# Autodesk Inventor assembly: Mark 4.5
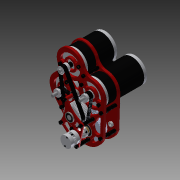
[picture p0: Inventor's stored thumbnail of the model, 180x180]
Saved by Autodesk Inventor 2013 (Build 170138000, 138)
## iProperties
Created: 2013-06-28
Part Number: Mark 4.5
Document SubType Name: Assembly
Designer: mvarma
Author: mvarma
## Documents named in this file (58)
- C:\Users\mvarma\Desktop\GRT 2013-2014 Gearbox\Mark 4\Mark 4.5.iam
- C:\Users\mvarma\Desktop\GRT 2013-2014 Gearbox\Mark 4\Plates\Mounting Plate.ipt
- C:\Users\mvarma\Desktop\GRT 2013-2014 Gearbox\Mark 4\Plates\Cim Plate.ipt
- C:\Users\mvarma\Desktop\GRT 2013-2014 Gearbox\Mark 4\Plates\Pnuematic Plate.ipt
- C:\Users\mvarma\Desktop\GRT 2013-2014 Gearbox\Mark 4\Plates\Main Connecting Standoff.ipt
- C:\Users\mvarma\Desktop\GRT 2013-2014 Gearbox\Mark 4\Pem Nuts\10-32 Clinch Style Pem Nut .091 Minimum Panel Thickness.ipt
- C:\Users\mvarma\Desktop\GRT 2013-2014 Gearbox\Mark 4\Pem Nuts\.25-20 Clinch Style Pem Nut .125 Minimum Panel Thickness.ipt
- C:\Users\mvarma\Desktop\GRT 2013-2014 Gearbox\Mark 4\Bearings\FR6-2ZZ - Hex.ipt
- C:\Users\mvarma\Desktop\GRT 2013-2014 Gearbox\Mark 4\Bearings\FR8-2RS.ipt
- C:\Users\mvarma\Desktop\GRT 2013-2014 Gearbox\Mark 4\Bearings\FR6-2RS.ipt
- C:\Users\mvarma\Desktop\GRT 2013-2014 Gearbox\Mark 4\Encoder\Encoder Mount.ipt
- C:\Users\mvarma\Desktop\GRT 2013-2014 Gearbox\Mark 4\Encoder\S4-120-250-N-S-B.ipt
- C:\Users\mvarma\Desktop\GRT 2013-2014 Gearbox\Mark 4\Shafts\Cluster Shaft.ipt
- C:\Users\mvarma\Desktop\GRT 2013-2014 Gearbox\Mark 4\Shafts\Flexible Shaft Coupler 6208K411.ipt
- C:\Users\mvarma\Desktop\GRT 2013-2014 Gearbox\Mark 4\Spacers\Cluster Shaft Spacer.ipt
- C:\Users\mvarma\Desktop\GRT 2013-2014 Gearbox\Mark 4\Gears\15T 20DP - .375 Hex Bore.ipt
- C:\Users\mvarma\Desktop\GRT 2013-2014 Gearbox\Mark 4\Gears\28T 20DP - .375 Hex Bore.ipt
- C:\Users\mvarma\Desktop\GRT 2013-2014 Gearbox\Mark 4\Shafts\Output Shaft.ipt
- C:\Users\mvarma\Desktop\GRT 2013-2014 Gearbox\Mark 4\Spacers\Shim 10 thou .500 Bore.ipt
- C:\Users\mvarma\Desktop\GRT 2013-2014 Gearbox\Mark 4\Bearings\R10-Open.ipt
- C:\Users\mvarma\Desktop\GRT 2013-2014 Gearbox\Mark 4\Gears\35T 20DP - .188 Ball Shifting Bore.ipt
- C:\Users\mvarma\Desktop\GRT 2013-2014 Gearbox\Mark 4\Gears\48T 20DP - .188 Ball Shifting Bore.ipt
- C:\Users\mvarma\Desktop\GRT 2013-2014 Gearbox\Mark 4\Bearings\Thrust Bearing Washer - .6250 Bore.ipt
- C:\Users\mvarma\Desktop\GRT 2013-2014 Gearbox\Mark 4\Spacers\Shim 10 thou .625 Bore.ipt
- C:\Users\mvarma\Desktop\GRT 2013-2014 Gearbox\Mark 4\Bolts\Socket Head Cap Screw 10-32 Thread 1.750 Length.ipt
- C:\Users\mvarma\Desktop\GRT 2013-2014 Gearbox\Mark 4\Plates\Supporting Plate Standoff.ipt
- C:\Users\mvarma\Desktop\GRT 2013-2014 Gearbox\Mark 4\Spacers\Shim 10 thou .375 Bore.ipt
- C:\Users\mvarma\Desktop\GRT 2013-2014 Gearbox\Mark 4\Pulleys\48T 3mm GT2 - .375 Hex Broach - Hubless.ipt
- C:\Users\mvarma\Desktop\GRT 2013-2014 Gearbox\Mark 4\Pem Nuts\4-40 Clinch Style Pem Nut .091 Minimum Panel Thickness.ipt
- C:\Users\mvarma\Desktop\GRT 2013-2014 Gearbox\Mark 4\Shafts\Tensioning Shaft.ipt
- C:\Users\mvarma\Desktop\GRT 2013-2014 Gearbox\Mark 4\Spacers\Belt Shaft Spacer 2.ipt
- C:\Users\mvarma\Desktop\GRT 2013-2014 Gearbox\Mark 4\Bearings\R4-2RS.ipt
- C:\Users\mvarma\Desktop\GRT 2013-2014 Gearbox\Mark 4\Bolts\Socket Head Cap Screw 10-32 Thread 1.500 Length.ipt
- C:\Users\mvarma\Desktop\GRT 2013-2014 Gearbox\Mark 4\Motors\CIM Can.ipt
- C:\Users\mvarma\Desktop\GRT 2013-2014 Gearbox\Mark 4\Motors\Mini CIM Can.ipt
- C:\Users\mvarma\Desktop\GRT 2013-2014 Gearbox\Mark 4\Motors\Rotor.ipt
- C:\Users\mvarma\Desktop\GRT 2013-2014 Gearbox\Mark 4\Bolts\Socket Head Cap Screw 10-32 Thread 3.000 Length.ipt
- C:\Users\mvarma\Desktop\GRT 2013-2014 Gearbox\Mark 4\Belts\267 mm Belt.ipt
- C:\Users\mvarma\Desktop\GRT 2013-2014 Gearbox\Mark 4\Belts\285 mm Belt.ipt
- C:\Users\mvarma\Desktop\GRT 2013-2014 Gearbox\Mark 4\Pulleys\16T 3mm GT2 - 8mm Key Broach.ipt
- C:\Users\mvarma\Desktop\GRT 2013-2014 Gearbox\Mark 4\Spacers\Cim Spacer.ipt
- C:\Users\mvarma\Desktop\GRT 2013-2014 Gearbox\Mark 4\Spacers\MiniCim Spacer.ipt
- C:\Users\mvarma\Desktop\GRT 2013-2014 Gearbox\Mark 4\Shafts\Ball Shifting Shaft.ipt
- C:\Users\mvarma\Desktop\GRT 2013-2014 Gearbox\Mark 4\Shafts\Output Shaft Insert.ipt
- C:\Users\mvarma\Desktop\GRT 2013-2014 Gearbox\Mark 4\Bearings\R3-2RS.ipt
- C:\Users\mvarma\Desktop\GRT 2013-2014 Gearbox\Mark 4\.0625 Spring Pin .2500 Long.ipt
- C:\Users\mvarma\Desktop\GRT 2013-2014 Gearbox\Mark 4\Pneumatic\Pneumatic Connector -Actuator Side.ipt
- C:\Users\mvarma\Desktop\GRT 2013-2014 Gearbox\Mark 4\Pneumatic\Pneumatic Connector -Shaft Side Cover.ipt
- C:\Users\mvarma\Desktop\GRT 2013-2014 Gearbox\Mark 4\Pneumatic\Pancake Pneumatic.iam
- C:\Users\mvarma\Desktop\GRT 2013-2014 Gearbox\Mark 4\Bolts\Button Head Cap Screw 4-40 Thread .125 Length.ipt
- C:\Users\mvarma\Desktop\GRT 2013-2014 Gearbox\Mark 4\Shafts\Output Shaft Hex Sleave.ipt
- C:\Users\mvarma\Desktop\GRT 2013-2014 Gearbox\Mark 4\Frame Segment.ipt
- C:\Users\mvarma\Desktop\GRT 2013-2014 Gearbox\Mark 4\Bolts\Socket Head Cap Screw 6-32 Thread 1.000 Length.ipt
- C:\Users\mvarma\Desktop\GRT 2013-2014 Gearbox\Mark 4\Plates\Cim Adjustment Block.ipt
- C:\Users\mvarma\Desktop\GRT 2013-2014 Gearbox\Mark 4\Bolts\Socket Head Cap Screw 6-32 Thread .500 Length.ipt
- C:\Users\mvarma\Desktop\GRT 2013-2014 Gearbox\Mark 4\Bolts\Socket Head Cap Screw 6-32 Thread .375 Length.ipt
- C:\Users\mvarma\Desktop\GRT 2013-2014 Gearbox\Mark 4\Bolts\Socket Head Cap Screw 10-32 Thread .750 Length.ipt
- C:\Users\mvarma\Desktop\GRT 2013-2014 Gearbox\Mark 4\Bolts\Socket Head Cap Screw 4-40 Thread 1.000 Length.ipt
## Components (110 placed, 57 different names)
1. Frame Segment:1 — Mate:228, Mate:229
2. Socket Head Cap Screw 4-40 Thread 1.000 Length:1 — Mate:270, Mate:272
3. Socket Head Cap Screw 4-40 Thread 1.000 Length:2 — Mate:271, Mate:273
4. 267 mm Belt:1 — Mate:174, Mate:175, Mate:179, Flush:2, Flush:3
5. 285 mm Belt:1 — Mate:176, Mate:177, Mate:178, Flush:1
6. Socket Head Cap Screw 6-32 Thread 1.000 Length:1 — Mate:232, Mate:234
7. Socket Head Cap Screw 6-32 Thread 1.000 Length:2 — Mate:231, Mate:233
8. S4-120-250-N-S-B:1 — Mate:66, Mate:67
9. Flexible Shaft Coupler 6208K411:1 — Mate:64, Mate:65, Mate:66, Mate:67
10. Encoder Mount:1 — Mate:225, Mate:226, Mate:227, Mate:231, Mate:232, Mate:233, Mate:234
11. Cim Spacer:1 — Mate:184, Mate:185
12. MiniCim Spacer:1 — Mate:187, Mate:188
13. Cim Spacer:2 — Mate:183, Mate:186
14. CIM Can:1 — Mate:153, Mate:154, Mate:155, Mate:163, Mate:166, Mate:185
15. CIM Can:2 — Mate:156, Mate:157, Mate:158, Mate:164, Mate:165, Mate:186
16. Mini CIM Can:1 — Mate:159, Mate:160, Mate:161, Mate:162, Mate:167, Mate:188, Mate:254
17. Rotor:1 — Mate:164, Mate:165, Mate:175, Mate:181, Mate:183
18. Rotor:2 — Mate:163, Mate:166, Mate:180, Mate:184
19. Rotor:3 — Mate:162, Mate:167, Mate:177, Mate:182, Mate:187
20. Socket Head Cap Screw 10-32 Thread .750 Length:1 — Mate:262, Mate:263
21. Socket Head Cap Screw 10-32 Thread .750 Length:2 — Mate:252, Mate:253
22. Socket Head Cap Screw 10-32 Thread .750 Length:3 — Mate:254, Mate:255
23. Socket Head Cap Screw 10-32 Thread .750 Length:4 — Mate:260, Mate:261
24. Socket Head Cap Screw 10-32 Thread .750 Length:5 — Mate:256, Mate:259
25. Socket Head Cap Screw 10-32 Thread .750 Length:6 — Mate:257, Mate:258
26. Pneumatic Connector -Actuator Side:1 — Mate:196, Mate:197, Mate:198, Mate:203, Mate:210, Mate:211
27. Pneumatic Connector -Shaft Side Cover:1 — Mate:196, Mate:197, Mate:198, Mate:201, Mate:214, Mate:219, Mate:220, Mate:221, Mate:222
28. Pancake Pneumatic:1 [sub-assembly] — Mate:209, Mate:210, Mate:211, Mate:212, Mate:213, Mate:270, Mate:271, Mate:272, Mate:273
29. Button Head Cap Screw 4-40 Thread .125 Length:1 — Mate:221, Mate:222
30. Button Head Cap Screw 4-40 Thread .125 Length:2 — Mate:219, Mate:220
31. 16T 3mm GT2 - 8mm Key Broach:1 — Mate:180, Flush:3
32. 16T 3mm GT2 - 8mm Key Broach:2 — Mate:181, Flush:2
33. 16T 3mm GT2 - 8mm Key Broach:3 — Mate:182, Flush:1
34. Supporting Plate Standoff:1 — Mate:117, Mate:120, Mate:122
35. Supporting Plate Standoff:2 — Mate:118, Mate:121
36. Supporting Plate Standoff:3 — Mate:116, Mate:119
37. Main Connecting Standoff:1 — Mate:10, Mate:28
38. Main Connecting Standoff:2 — Mate:11, Mate:29
39. Main Connecting Standoff:3 — Mate:3, Mate:12, Mate:27, Mate:140
40. Main Connecting Standoff:4 — Mate:15, Mate:26
41. Main Connecting Standoff:5 — Mate:5, Mate:16, Mate:25
42. Main Connecting Standoff:6 — Mate:17, Mate:23
43. Main Connecting Standoff:7 — Mate:20, Mate:21
44. Main Connecting Standoff:8 — Mate:8, Mate:19, Mate:24
45. Main Connecting Standoff:9 — Mate:18, Mate:22, Mate:206
46. Mounting Plate:1 — Mate:3, Mate:5, Mate:8, Mate:21, Mate:22, Mate:23, Mate:24, Mate:25, Mate:26, Mate:27, Mate:28, Mate:29, Mate:31, Mate:34, Mate:36, Mate:39, Mate:40, Mate:41, Mate:42, Mate:43, Mate:44, Mate:45, Mate:46, Mate:47, Mate:48, Mate:49, Mate:50, Mate:51, Mate:53, Mate:55, Mate:56, Mate:57, Mate:68, Mate:73, Mate:74, Mate:225, Mate:226, Mate:227, Mate:229, Mate:235, Mate:236, Mate:237, Mate:243, Mate:244, Mate:245, Mate:264, Mate:265, Mate:266, Mate:267, Mate:268, Mate:269
47. FR8-2RS:1 — Mate:53, Mate:55, Mate:80, Mate:83
48. FR6-2RS:1 — Mate:56, Mate:57, Mate:72
49. Cim Plate:1 — Mate:10, Mate:11, Mate:12, Mate:15, Mate:16, Mate:17, Mate:18, Mate:19, Mate:20, Mate:58, Mate:59, Mate:60, Mate:61, Mate:102, Mate:103, Mate:104, Mate:105, Mate:106, Mate:107, Mate:108, Mate:109, Mate:110, Mate:111, Mate:112, Mate:113, Mate:114, Mate:115, Mate:116, Mate:117, Mate:118, Mate:119, Mate:120, Mate:121, Mate:139, Mate:140, Mate:141, Mate:142, Mate:153, Mate:154, Mate:155, Mate:156, Mate:157, Mate:158, Mate:159, Mate:160, Mate:161, Mate:174, Mate:176, Mate:206, Mate:252, Mate:253, Mate:255, Mate:256, Mate:257, Mate:258, Mate:259, Mate:260, Mate:261, Mate:262, Mate:263
50. FR6-2ZZ - Hex:1 — Mate:60, Mate:61, Mate:79, Mate:125
51. FR8-2RS:2 — Mate:58, Mate:59, Mate:214
52. Socket Head Cap Screw 10-32 Thread 1.500 Length:1 — Mate:151, Mate:152
53. Pnuematic Plate:1 — Mate:114, Mate:115, Mate:122, Mate:133, Mate:134, Mate:139, Mate:146, Mate:151, Mate:152, Mate:168, Mate:169, Mate:170, Mate:171, Mate:172, Mate:173, Mate:209, Mate:212, Mate:213, Mate:215, Mate:216, Mate:217, Mate:218
54. FR6-2RS:2 — Mate:133, Mate:134
55. Socket Head Cap Screw 10-32 Thread 3.000 Length:1 — Mate:170, Mate:173
56. Socket Head Cap Screw 10-32 Thread 3.000 Length:2 — Mate:169, Mate:171
57. Socket Head Cap Screw 10-32 Thread 3.000 Length:3 — Mate:168, Mate:172
58. Ball Shifting Shaft:1 — Mate:191, Mate:192, Mate:193, Mate:194, Mate:195, Mate:201
59. R3-2RS:1 — Mate:192, Mate:193, Mate:203
60. .0625 Spring Pin .2500 Long:1 — Mate:194, Mate:195
61. Cluster Shaft:1 — Mate:64, Mate:65, Mate:68, Mate:71, Mate:75, Mate:76, Mate:79, Mate:123, Mate:124, Mate:126, Mate:127, Mate:128, Mate:129
62. Cluster Shaft Spacer:1 — Mate:71, Mate:72, Mate:78
63. 15T 20DP - .375 Hex Bore:1 — Mate:74, Mate:76, Mate:77
64. 28T 20DP - .375 Hex Bore:1 — Mate:73, Mate:75, Mate:77, Mate:78
65. Shim 10 thou .375 Bore:1 — Mate:123, Mate:132
66. Shim 10 thou .500 Bore:2 — Mate:124, Mate:125, Mate:131
67. 48T 3mm GT2 - .375 Hex Broach - Hubless:1 — Mate:126, Mate:128, Mate:130, Mate:132, Mate:178
68. 48T 3mm GT2 - .375 Hex Broach - Hubless:2 — Mate:127, Mate:129, Mate:130, Mate:131, Mate:179
69. Output Shaft Insert:1 — Mate:189, Mate:190, Mate:191
70. Shim 10 thou .625 Bore:1 — Mate:96, Mate:97
71. Thrust Bearing Washer - .6250 Bore:2 — Mate:94, Mate:95, Mate:97
72. 48T 20DP - .188 Ball Shifting Bore:1 — Mate:92, Mate:93, Mate:95
73. R10-Open:1 — Mate:90, Mate:91, Mate:93
74. Thrust Bearing Washer - .6250 Bore:1 — Mate:88, Mate:89, Mate:91
75. 35T 20DP - .188 Ball Shifting Bore:1 — Mate:86, Mate:87, Mate:89
76. R10-Open:2 — Mate:84, Mate:85, Mate:87
77. Shim 10 thou .500 Bore:1 — Mate:81, Mate:82, Mate:83, Mate:85
78. Output Shaft:1 — Mate:80, Mate:81, Mate:82, Mate:84, Mate:86, Mate:88, Mate:90, Mate:92, Mate:94, Mate:96, Mate:189, Mate:190, Mate:223, Mate:224, Flush:4, Mate:228
79. Output Shaft Hex Sleave:1 — Mate:223, Mate:224, Flush:4
80. Tensioning Shaft:1 — Mate:141, Mate:142, Mate:143, Mate:149
81. Belt Shaft Spacer 2:1 — Mate:143, Mate:146, Mate:150
82. R4-2RS:1 — Mate:147, Mate:148, Mate:149, Mate:150
83. R4-2RS:2 — Mate:147, Mate:148
84. Cim Adjustment Block:1 — Mate:235, Mate:236, Mate:237, Mate:238, Mate:239, Mate:240, Mate:241, Mate:251
85. Cim Adjustment Block:2 — Mate:243, Mate:244, Mate:245, Mate:246, Mate:247, Mate:248, Mate:249, Mate:250
86. Socket Head Cap Screw 6-32 Thread .500 Length:1 — Mate:239, Mate:240
87. Socket Head Cap Screw 6-32 Thread .500 Length:2 — Mate:238, Mate:241
88. Socket Head Cap Screw 6-32 Thread .375 Length:2 — Mate:251
89. Socket Head Cap Screw 6-32 Thread .500 Length:4 — Mate:246, Mate:249
90. Socket Head Cap Screw 6-32 Thread .500 Length:5 — Mate:247, Mate:248
91. Socket Head Cap Screw 6-32 Thread .375 Length:1 — Mate:250
92. 10-32 Clinch Style Pem Nut .091 Minimum Panel Thickness:1 — Mate:41, Mate:268
93. 10-32 Clinch Style Pem Nut .091 Minimum Panel Thickness:2 — Mate:34, Mate:40
94. 10-32 Clinch Style Pem Nut .091 Minimum Panel Thickness:3 — Mate:39, Mate:267
95. 10-32 Clinch Style Pem Nut .091 Minimum Panel Thickness:4 — Mate:31, Mate:42
96. 10-32 Clinch Style Pem Nut .091 Minimum Panel Thickness:5 — Mate:43, Mate:266
97. 10-32 Clinch Style Pem Nut .091 Minimum Panel Thickness:6 — Mate:44, Mate:265
98. 10-32 Clinch Style Pem Nut .091 Minimum Panel Thickness:7 — Mate:47, Mate:269
99. 10-32 Clinch Style Pem Nut .091 Minimum Panel Thickness:8 — Mate:36, Mate:45
100. 10-32 Clinch Style Pem Nut .091 Minimum Panel Thickness:9 — Mate:46, Mate:264
101. .25-20 Clinch Style Pem Nut .125 Minimum Panel Thickness:1 — Mate:49, Mate:50
102. .25-20 Clinch Style Pem Nut .125 Minimum Panel Thickness:2 — Mate:48, Mate:51
103. Socket Head Cap Screw 10-32 Thread 1.750 Length:4 — Mate:108, Mate:109
104. Socket Head Cap Screw 10-32 Thread 1.750 Length:5 — Mate:111, Mate:113
105. Socket Head Cap Screw 10-32 Thread 1.750 Length:6 — Mate:110, Mate:112
106. Socket Head Cap Screw 10-32 Thread 1.750 Length:7 — Mate:105, Mate:106
107. Socket Head Cap Screw 10-32 Thread 1.750 Length:8 — Mate:104, Mate:107
108. Socket Head Cap Screw 10-32 Thread 1.750 Length:9 — Mate:102, Mate:103
109. 4-40 Clinch Style Pem Nut .091 Minimum Panel Thickness:1 — Mate:216, Mate:218
110. 4-40 Clinch Style Pem Nut .091 Minimum Panel Thickness:2 — Mate:215, Mate:217
## Relationships (240: Mate 234, Flush 4, Tangent 2)
- Mate:3: Main Connecting Standoff:3 ↔ Mounting Plate:1
- Mate:5: Main Connecting Standoff:5 ↔ Mounting Plate:1
- Mate:8: Main Connecting Standoff:8 ↔ Mounting Plate:1
- Mate:10: Main Connecting Standoff:1 ↔ Cim Plate:1
- Mate:11: Main Connecting Standoff:2 ↔ Cim Plate:1
- Mate:12: Main Connecting Standoff:3 ↔ Cim Plate:1
- Mate:15: Main Connecting Standoff:4 ↔ Cim Plate:1
- Mate:16: Main Connecting Standoff:5 ↔ Cim Plate:1
- Mate:17: Main Connecting Standoff:6 ↔ Cim Plate:1
- Mate:18: Main Connecting Standoff:9 ↔ Cim Plate:1
- Mate:19: Main Connecting Standoff:8 ↔ Cim Plate:1
- Mate:20: Main Connecting Standoff:7 ↔ Cim Plate:1
- Mate:21: Main Connecting Standoff:7 ↔ Mounting Plate:1
- Mate:22: Main Connecting Standoff:9 ↔ Mounting Plate:1
- Mate:23: Main Connecting Standoff:6 ↔ Mounting Plate:1
- Mate:24: Main Connecting Standoff:8 ↔ Mounting Plate:1
- Mate:25: Main Connecting Standoff:5 ↔ Mounting Plate:1
- Mate:26: Main Connecting Standoff:4 ↔ Mounting Plate:1
- Mate:27: Main Connecting Standoff:3 ↔ Mounting Plate:1
- Mate:28: Main Connecting Standoff:1 ↔ Mounting Plate:1
- Mate:29: Main Connecting Standoff:2 ↔ Mounting Plate:1
- Mate:31: Mounting Plate:1 ↔ 10-32 Clinch Style Pem Nut .091 Minimum Panel Thickness:4
- Mate:34: Mounting Plate:1 ↔ 10-32 Clinch Style Pem Nut .091 Minimum Panel Thickness:2
- Mate:36: Mounting Plate:1 ↔ 10-32 Clinch Style Pem Nut .091 Minimum Panel Thickness:8
- Mate:39: Mounting Plate:1 ↔ 10-32 Clinch Style Pem Nut .091 Minimum Panel Thickness:3
- Mate:40: Mounting Plate:1 ↔ 10-32 Clinch Style Pem Nut .091 Minimum Panel Thickness:2
- Mate:41: Mounting Plate:1 ↔ 10-32 Clinch Style Pem Nut .091 Minimum Panel Thickness:1
- Mate:42: Mounting Plate:1 ↔ 10-32 Clinch Style Pem Nut .091 Minimum Panel Thickness:4
- Mate:43: Mounting Plate:1 ↔ 10-32 Clinch Style Pem Nut .091 Minimum Panel Thickness:5
- Mate:44: Mounting Plate:1 ↔ 10-32 Clinch Style Pem Nut .091 Minimum Panel Thickness:6
- Mate:45: Mounting Plate:1 ↔ 10-32 Clinch Style Pem Nut .091 Minimum Panel Thickness:8
- Mate:46: Mounting Plate:1 ↔ 10-32 Clinch Style Pem Nut .091 Minimum Panel Thickness:9
- Mate:47: Mounting Plate:1 ↔ 10-32 Clinch Style Pem Nut .091 Minimum Panel Thickness:7
- Mate:48: Mounting Plate:1 ↔ .25-20 Clinch Style Pem Nut .125 Minimum Panel Thickness:2
- Mate:49: Mounting Plate:1 ↔ .25-20 Clinch Style Pem Nut .125 Minimum Panel Thickness:1
- Mate:50: Mounting Plate:1 ↔ .25-20 Clinch Style Pem Nut .125 Minimum Panel Thickness:1
- Mate:51: Mounting Plate:1 ↔ .25-20 Clinch Style Pem Nut .125 Minimum Panel Thickness:2
- Mate:53: Mounting Plate:1 ↔ FR8-2RS:1
- Mate:55: Mounting Plate:1 ↔ FR8-2RS:1
- Mate:56: Mounting Plate:1 ↔ FR6-2RS:1
- Mate:57: Mounting Plate:1 ↔ FR6-2RS:1
- Mate:58: Cim Plate:1 ↔ FR8-2RS:2
- Mate:59: Cim Plate:1 ↔ FR8-2RS:2
- Mate:60: Cim Plate:1 ↔ FR6-2ZZ - Hex:1
- Mate:61: Cim Plate:1 ↔ FR6-2ZZ - Hex:1
- Mate:64: Flexible Shaft Coupler 6208K411:1 ↔ Cluster Shaft:1
- Mate:65: Flexible Shaft Coupler 6208K411:1 ↔ Cluster Shaft:1
- Mate:66: S4-120-250-N-S-B:1 ↔ Flexible Shaft Coupler 6208K411:1
- Mate:67: S4-120-250-N-S-B:1 ↔ Flexible Shaft Coupler 6208K411:1
- Mate:68: Mounting Plate:1 ↔ Cluster Shaft:1
- Mate:71: Cluster Shaft:1 ↔ Cluster Shaft Spacer:1
- Mate:72: FR6-2RS:1 ↔ Cluster Shaft Spacer:1
- Mate:73: Mounting Plate:1 ↔ 28T 20DP - .375 Hex Bore:1
- Mate:74: Mounting Plate:1 ↔ 15T 20DP - .375 Hex Bore:1
- Mate:75: Cluster Shaft:1 ↔ 28T 20DP - .375 Hex Bore:1
- Mate:76: Cluster Shaft:1 ↔ 15T 20DP - .375 Hex Bore:1
- Mate:77: 15T 20DP - .375 Hex Bore:1 ↔ 28T 20DP - .375 Hex Bore:1
- Mate:78: Cluster Shaft Spacer:1 ↔ 28T 20DP - .375 Hex Bore:1
- Mate:79: FR6-2ZZ - Hex:1 ↔ Cluster Shaft:1
- Mate:80: FR8-2RS:1 ↔ Output Shaft:1
- Mate:81: Shim 10 thou .500 Bore:1 ↔ Output Shaft:1
- Mate:82: Shim 10 thou .500 Bore:1 ↔ Output Shaft:1
- Mate:83: FR8-2RS:1 ↔ Shim 10 thou .500 Bore:1
- Mate:84: R10-Open:2 ↔ Output Shaft:1
- Mate:85: R10-Open:2 ↔ Shim 10 thou .500 Bore:1
- Mate:86: 35T 20DP - .188 Ball Shifting Bore:1 ↔ Output Shaft:1
- Mate:87: 35T 20DP - .188 Ball Shifting Bore:1 ↔ R10-Open:2
- Mate:88: Thrust Bearing Washer - .6250 Bore:1 ↔ Output Shaft:1
- Mate:89: Thrust Bearing Washer - .6250 Bore:1 ↔ 35T 20DP - .188 Ball Shifting Bore:1
- Mate:90: R10-Open:1 ↔ Output Shaft:1
- Mate:91: R10-Open:1 ↔ Thrust Bearing Washer - .6250 Bore:1
- Mate:92: 48T 20DP - .188 Ball Shifting Bore:1 ↔ Output Shaft:1
- Mate:93: 48T 20DP - .188 Ball Shifting Bore:1 ↔ R10-Open:1
- Mate:94: Thrust Bearing Washer - .6250 Bore:2 ↔ Output Shaft:1
- Mate:95: Thrust Bearing Washer - .6250 Bore:2 ↔ 48T 20DP - .188 Ball Shifting Bore:1
- Mate:96: Shim 10 thou .625 Bore:1 ↔ Output Shaft:1
- Mate:97: Shim 10 thou .625 Bore:1 ↔ Thrust Bearing Washer - .6250 Bore:2
- Mate:102: Cim Plate:1 ↔ Socket Head Cap Screw 10-32 Thread 1.750 Length:9
- Mate:103: Cim Plate:1 ↔ Socket Head Cap Screw 10-32 Thread 1.750 Length:9
- Mate:104: Cim Plate:1 ↔ Socket Head Cap Screw 10-32 Thread 1.750 Length:8
- Mate:105: Cim Plate:1 ↔ Socket Head Cap Screw 10-32 Thread 1.750 Length:7
- Mate:106: Cim Plate:1 ↔ Socket Head Cap Screw 10-32 Thread 1.750 Length:7
- Mate:107: Cim Plate:1 ↔ Socket Head Cap Screw 10-32 Thread 1.750 Length:8
- Mate:108: Cim Plate:1 ↔ Socket Head Cap Screw 10-32 Thread 1.750 Length:4
- Mate:109: Cim Plate:1 ↔ Socket Head Cap Screw 10-32 Thread 1.750 Length:4
- Mate:110: Cim Plate:1 ↔ Socket Head Cap Screw 10-32 Thread 1.750 Length:6
- Mate:111: Cim Plate:1 ↔ Socket Head Cap Screw 10-32 Thread 1.750 Length:5
- Mate:112: Cim Plate:1 ↔ Socket Head Cap Screw 10-32 Thread 1.750 Length:6
- Mate:113: Cim Plate:1 ↔ Socket Head Cap Screw 10-32 Thread 1.750 Length:5
- Mate:114: Cim Plate:1 ↔ Pnuematic Plate:1
- Mate:115: Cim Plate:1 ↔ Pnuematic Plate:1
- Mate:116: Supporting Plate Standoff:3 ↔ Cim Plate:1
- Mate:117: Supporting Plate Standoff:1 ↔ Cim Plate:1
- Mate:118: Supporting Plate Standoff:2 ↔ Cim Plate:1
- Mate:119: Supporting Plate Standoff:3 ↔ Cim Plate:1
- Mate:120: Supporting Plate Standoff:1 ↔ Cim Plate:1
- Mate:121: Supporting Plate Standoff:2 ↔ Cim Plate:1
- Mate:122: Supporting Plate Standoff:1 ↔ Pnuematic Plate:1
- Mate:123: Cluster Shaft:1 ↔ Shim 10 thou .375 Bore:1
- Mate:124: Cluster Shaft:1 ↔ Shim 10 thou .500 Bore:2
- Mate:125: FR6-2ZZ - Hex:1 ↔ Shim 10 thou .500 Bore:2
- Mate:126: Cluster Shaft:1 ↔ 48T 3mm GT2 - .375 Hex Broach - Hubless:1
- Mate:127: Cluster Shaft:1 ↔ 48T 3mm GT2 - .375 Hex Broach - Hubless:2
- Mate:128: Cluster Shaft:1 ↔ 48T 3mm GT2 - .375 Hex Broach - Hubless:1
- Mate:129: Cluster Shaft:1 ↔ 48T 3mm GT2 - .375 Hex Broach - Hubless:2
- Mate:130: 48T 3mm GT2 - .375 Hex Broach - Hubless:1 ↔ 48T 3mm GT2 - .375 Hex Broach - Hubless:2
- Mate:131: Shim 10 thou .500 Bore:2 ↔ 48T 3mm GT2 - .375 Hex Broach - Hubless:2
- Mate:132: Shim 10 thou .375 Bore:1 ↔ 48T 3mm GT2 - .375 Hex Broach - Hubless:1
- Mate:133: Pnuematic Plate:1 ↔ FR6-2RS:2
- Mate:134: Pnuematic Plate:1 ↔ FR6-2RS:2
- Mate:139: Cim Plate:1 ↔ Pnuematic Plate:1
- Mate:140: Main Connecting Standoff:3 ↔ Cim Plate:1
- Mate:141: Cim Plate:1 ↔ Tensioning Shaft:1
- Mate:142: Cim Plate:1 ↔ Tensioning Shaft:1
- Mate:143: Tensioning Shaft:1 ↔ Belt Shaft Spacer 2:1
- Mate:146: Pnuematic Plate:1 ↔ Belt Shaft Spacer 2:1
- Mate:147: R4-2RS:1 ↔ R4-2RS:2
- Mate:148: R4-2RS:1 ↔ R4-2RS:2
- Mate:149: Tensioning Shaft:1 ↔ R4-2RS:1
- Mate:150: Belt Shaft Spacer 2:1 ↔ R4-2RS:1
- Mate:151: Socket Head Cap Screw 10-32 Thread 1.500 Length:1 ↔ Pnuematic Plate:1
- Mate:152: Socket Head Cap Screw 10-32 Thread 1.500 Length:1 ↔ Pnuematic Plate:1
- Mate:153: CIM Can:1 ↔ Cim Plate:1
- Mate:154: CIM Can:1 ↔ Cim Plate:1
- Mate:155: CIM Can:1 ↔ Cim Plate:1
- Mate:156: CIM Can:2 ↔ Cim Plate:1
- Mate:157: CIM Can:2 ↔ Cim Plate:1
- Mate:158: CIM Can:2 ↔ Cim Plate:1
- Mate:159: Mini CIM Can:1 ↔ Cim Plate:1
- Mate:160: Mini CIM Can:1 ↔ Cim Plate:1
- Mate:161: Mini CIM Can:1 ↔ Cim Plate:1
- Mate:162: Mini CIM Can:1 ↔ Rotor:3
- Mate:163: CIM Can:1 ↔ Rotor:2
- Mate:164: CIM Can:2 ↔ Rotor:1
- Mate:165: CIM Can:2 ↔ Rotor:1
- Mate:166: CIM Can:1 ↔ Rotor:2
- Mate:167: Mini CIM Can:1 ↔ Rotor:3
- Mate:168: Pnuematic Plate:1 ↔ Socket Head Cap Screw 10-32 Thread 3.000 Length:3
- Mate:169: Pnuematic Plate:1 ↔ Socket Head Cap Screw 10-32 Thread 3.000 Length:2
- Mate:170: Pnuematic Plate:1 ↔ Socket Head Cap Screw 10-32 Thread 3.000 Length:1
- Mate:171: Pnuematic Plate:1 ↔ Socket Head Cap Screw 10-32 Thread 3.000 Length:2
- Mate:172: Pnuematic Plate:1 ↔ Socket Head Cap Screw 10-32 Thread 3.000 Length:3
- Mate:173: Pnuematic Plate:1 ↔ Socket Head Cap Screw 10-32 Thread 3.000 Length:1
- Mate:174: 267 mm Belt:1 ↔ Cim Plate:1
- Mate:175: 267 mm Belt:1 ↔ Rotor:1
- Mate:176: 285 mm Belt:1 ↔ Cim Plate:1
- Mate:177: 285 mm Belt:1 ↔ Rotor:3
- Mate:178: 285 mm Belt:1 ↔ 48T 3mm GT2 - .375 Hex Broach - Hubless:1
- Mate:179: 267 mm Belt:1 ↔ 48T 3mm GT2 - .375 Hex Broach - Hubless:2
- Mate:180: Rotor:2 ↔ 16T 3mm GT2 - 8mm Key Broach:1
- Mate:181: Rotor:1 ↔ 16T 3mm GT2 - 8mm Key Broach:2
- Mate:182: Rotor:3 ↔ 16T 3mm GT2 - 8mm Key Broach:3
- Flush:1: 285 mm Belt:1 ↔ 16T 3mm GT2 - 8mm Key Broach:3
- Flush:2: 267 mm Belt:1 ↔ 16T 3mm GT2 - 8mm Key Broach:2
- Flush:3: 267 mm Belt:1 ↔ 16T 3mm GT2 - 8mm Key Broach:1
- Mate:183: Cim Spacer:2 ↔ Rotor:1
- Mate:184: Cim Spacer:1 ↔ Rotor:2
- Mate:185: Cim Spacer:1 ↔ CIM Can:1
- Mate:186: Cim Spacer:2 ↔ CIM Can:2
- Mate:187: MiniCim Spacer:1 ↔ Rotor:3
- Mate:188: MiniCim Spacer:1 ↔ Mini CIM Can:1
- Mate:189: Output Shaft Insert:1 ↔ Output Shaft:1
- Mate:190: Output Shaft Insert:1 ↔ Output Shaft:1
- Mate:191: Ball Shifting Shaft:1 ↔ Output Shaft Insert:1
- Mate:192: Ball Shifting Shaft:1 ↔ R3-2RS:1
- Mate:193: Ball Shifting Shaft:1 ↔ R3-2RS:1
- Mate:194: Ball Shifting Shaft:1 ↔ .0625 Spring Pin .2500 Long:1
- Mate:195: Ball Shifting Shaft:1 ↔ .0625 Spring Pin .2500 Long:1
- Mate:196: Pneumatic Connector -Actuator Side:1 ↔ Pneumatic Connector -Shaft Side Cover:1
- Mate:197: Pneumatic Connector -Actuator Side:1 ↔ Pneumatic Connector -Shaft Side Cover:1
- Mate:198: Pneumatic Connector -Actuator Side:1 ↔ Pneumatic Connector -Shaft Side Cover:1
- Mate:201: Pneumatic Connector -Shaft Side Cover:1 ↔ Ball Shifting Shaft:1
- Mate:203: Pneumatic Connector -Actuator Side:1 ↔ R3-2RS:1
- Mate:206: Main Connecting Standoff:9 ↔ Cim Plate:1
- Mate:209: Pancake Pneumatic:1 ↔ Pnuematic Plate:1
- Mate:210: Pneumatic Connector -Actuator Side:1 ↔ Pancake Pneumatic:1
- Mate:211: Pneumatic Connector -Actuator Side:1 ↔ Pancake Pneumatic:1
- Mate:212: Pancake Pneumatic:1 ↔ Pnuematic Plate:1
- Mate:213: Pancake Pneumatic:1 ↔ Pnuematic Plate:1
- Mate:214 (8.8582 mm): Pneumatic Connector -Shaft Side Cover:1 ↔ FR8-2RS:2
- Mate:215: Pnuematic Plate:1 ↔ 4-40 Clinch Style Pem Nut .091 Minimum Panel Thickness:2
- Mate:216: Pnuematic Plate:1 ↔ 4-40 Clinch Style Pem Nut .091 Minimum Panel Thickness:1
- Mate:217: Pnuematic Plate:1 ↔ 4-40 Clinch Style Pem Nut .091 Minimum Panel Thickness:2
- Mate:218: Pnuematic Plate:1 ↔ 4-40 Clinch Style Pem Nut .091 Minimum Panel Thickness:1
- Mate:219: Pneumatic Connector -Shaft Side Cover:1 ↔ Button Head Cap Screw 4-40 Thread .125 Length:2
- Mate:220: Pneumatic Connector -Shaft Side Cover:1 ↔ Button Head Cap Screw 4-40 Thread .125 Length:2
- Mate:221: Pneumatic Connector -Shaft Side Cover:1 ↔ Button Head Cap Screw 4-40 Thread .125 Length:1
- Mate:222: Pneumatic Connector -Shaft Side Cover:1 ↔ Button Head Cap Screw 4-40 Thread .125 Length:1
- Mate:223: Output Shaft:1 ↔ Output Shaft Hex Sleave:1
- Mate:224: Output Shaft:1 ↔ Output Shaft Hex Sleave:1
- Flush:4: Output Shaft:1 ↔ Output Shaft Hex Sleave:1
- Mate:225: Encoder Mount:1 ↔ Mounting Plate:1
- Mate:226: Encoder Mount:1 ↔ Mounting Plate:1
- Mate:227: Encoder Mount:1 ↔ Mounting Plate:1
- Mate:228: Frame Segment:1 ↔ Output Shaft:1
- Mate:229: Frame Segment:1 ↔ Mounting Plate:1
- Mate:231: Socket Head Cap Screw 6-32 Thread 1.000 Length:2 ↔ Encoder Mount:1
- Mate:232: Socket Head Cap Screw 6-32 Thread 1.000 Length:1 ↔ Encoder Mount:1
- Mate:233: Socket Head Cap Screw 6-32 Thread 1.000 Length:2 ↔ Encoder Mount:1
- Mate:234: Socket Head Cap Screw 6-32 Thread 1.000 Length:1 ↔ Encoder Mount:1
- Mate:235: Mounting Plate:1 ↔ Cim Adjustment Block:1
- Mate:236: Mounting Plate:1 ↔ Cim Adjustment Block:1
- Mate:237: Mounting Plate:1 ↔ Cim Adjustment Block:1
- Mate:238: Cim Adjustment Block:1 ↔ Socket Head Cap Screw 6-32 Thread .500 Length:2
- Mate:239: Cim Adjustment Block:1 ↔ Socket Head Cap Screw 6-32 Thread .500 Length:1
- Mate:240: Cim Adjustment Block:1 ↔ Socket Head Cap Screw 6-32 Thread .500 Length:1
- Mate:241: Cim Adjustment Block:1 ↔ Socket Head Cap Screw 6-32 Thread .500 Length:2
- [Tangent]: CIM Can:2 ↔ Socket Head Cap Screw 6-32 Thread .375 Length:2
- Mate:243: Mounting Plate:1 ↔ Cim Adjustment Block:2
- Mate:244: Mounting Plate:1 ↔ Cim Adjustment Block:2
- Mate:245: Mounting Plate:1 ↔ Cim Adjustment Block:2
- Mate:246: Cim Adjustment Block:2 ↔ Socket Head Cap Screw 6-32 Thread .500 Length:4
- Mate:247: Cim Adjustment Block:2 ↔ Socket Head Cap Screw 6-32 Thread .500 Length:5
- Mate:248: Cim Adjustment Block:2 ↔ Socket Head Cap Screw 6-32 Thread .500 Length:5
- Mate:249: Cim Adjustment Block:2 ↔ Socket Head Cap Screw 6-32 Thread .500 Length:4
- [Tangent]: Mini CIM Can:1 ↔ Socket Head Cap Screw 6-32 Thread .375 Length:1
- Mate:250: Cim Adjustment Block:2 ↔ Socket Head Cap Screw 6-32 Thread .375 Length:1
- Mate:251: Cim Adjustment Block:1 ↔ Socket Head Cap Screw 6-32 Thread .375 Length:2
- Mate:252: Socket Head Cap Screw 10-32 Thread .750 Length:2 ↔ Cim Plate:1
- Mate:253: Socket Head Cap Screw 10-32 Thread .750 Length:2 ↔ Cim Plate:1
- Mate:254: Mini CIM Can:1 ↔ Socket Head Cap Screw 10-32 Thread .750 Length:3
- Mate:255: Socket Head Cap Screw 10-32 Thread .750 Length:3 ↔ Cim Plate:1
- Mate:256: Socket Head Cap Screw 10-32 Thread .750 Length:5 ↔ Cim Plate:1
- Mate:257: Socket Head Cap Screw 10-32 Thread .750 Length:6 ↔ Cim Plate:1
- Mate:258: Socket Head Cap Screw 10-32 Thread .750 Length:6 ↔ Cim Plate:1
- Mate:259: Socket Head Cap Screw 10-32 Thread .750 Length:5 ↔ Cim Plate:1
- Mate:260: Socket Head Cap Screw 10-32 Thread .750 Length:4 ↔ Cim Plate:1
- Mate:261: Socket Head Cap Screw 10-32 Thread .750 Length:4 ↔ Cim Plate:1
- Mate:262: Socket Head Cap Screw 10-32 Thread .750 Length:1 ↔ Cim Plate:1
- Mate:263: Socket Head Cap Screw 10-32 Thread .750 Length:1 ↔ Cim Plate:1
- Mate:264: Mounting Plate:1 ↔ 10-32 Clinch Style Pem Nut .091 Minimum Panel Thickness:9
- Mate:265: Mounting Plate:1 ↔ 10-32 Clinch Style Pem Nut .091 Minimum Panel Thickness:6
- Mate:266: Mounting Plate:1 ↔ 10-32 Clinch Style Pem Nut .091 Minimum Panel Thickness:5
- Mate:267: Mounting Plate:1 ↔ 10-32 Clinch Style Pem Nut .091 Minimum Panel Thickness:3
- Mate:268: Mounting Plate:1 ↔ 10-32 Clinch Style Pem Nut .091 Minimum Panel Thickness:1
- Mate:269: Mounting Plate:1 ↔ 10-32 Clinch Style Pem Nut .091 Minimum Panel Thickness:7
- Mate:270: Socket Head Cap Screw 4-40 Thread 1.000 Length:1 ↔ Pancake Pneumatic:1
- Mate:271: Socket Head Cap Screw 4-40 Thread 1.000 Length:2 ↔ Pancake Pneumatic:1
- Mate:272: Socket Head Cap Screw 4-40 Thread 1.000 Length:1 ↔ Pancake Pneumatic:1
- Mate:273: Socket Head Cap Screw 4-40 Thread 1.000 Length:2 ↔ Pancake Pneumatic:1
